# Autodesk Inventor assembly: TestAssem
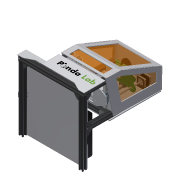
[picture p0: Inventor's stored thumbnail of the model, 180x180]
Saved by Autodesk Inventor 2014 (Build 180170000, 170)
## iProperties
Created: 2015-01-19
Part Number: TestAssem
Document SubType Name: Assembly
Designer: Peele
Author: Peele
## Documents named in this file (21)
- E:\Copy\DLP\PandaPrint\SubAssem\TestAssem.iam
- E:\Copy\DLP\PandaPrint\SubAssem\InnerTopAssem.iam
- E:\Copy\DLP\PandaPrint\SubAssem\NewVatAssem.iam
- E:\Copy\DLP\PandaPrint\CustomParts\InnerFront.ipt
- E:\Copy\DLP\PandaPrint\CustomParts\InnerSide.ipt
- E:\Copy\DLP\PandaPrint\SubAssem\NewFrame.iam
- E:\Copy\DLP\PandaPrint\CustomParts\ProjectorPlate.ipt
- E:\Copy\DLP\PandaPrint\StockParts\Projector-AcerP1500.ipt
- E:\Copy\DLP\PandaPrint\CustomParts\MirrorPlate.ipt
- E:\Copy\DLP\PandaPrint\SubAssem\StepperWithMount.iam
- E:\Copy\DLP\PandaPrint\CustomParts\BackPlate.ipt
- E:\Copy\DLP\PandaPrint\StockParts\Rail.ipt
- E:\Copy\DLP\PandaPrint\SubAssem\PlatformAssenm.iam
- E:\Copy\DLP\PandaPrint\StockParts\bLOCK.ipt
- E:\Copy\DLP\PandaPrint\CustomParts\BottomRightSide.ipt
- E:\Copy\DLP\PandaPrint\SubAssem\FrontCover.iam
- E:\Copy\DLP\PandaPrint\CustomParts\LeftSidePanel.ipt
- E:\Copy\DLP\PandaPrint\CustomParts\FrontPanel.ipt
- E:\Copy\DLP\PandaPrint\CustomParts\ControlRightPanel.ipt
- E:\Copy\DLP\PandaPrint\StockParts\Rail\Rail-02.ipt
- E:\Copy\DLP\PandaPrint\CustomParts\ControlPanel.ipt
## Components (21 placed, 19 different names)
1. InnerTopAssem:1 [sub-assembly] — Mate:1, Flush:1, Mate:2, Mate:3, Mate:4, Flush:2, Mate:5, Mate:10, Flush:7, Flush:13, Mate:27, Mate:31, Mate:44, Flush:28, Mate:49
2. NewVatAssem:1 [sub-assembly] — Mate:3, Mate:4, Mate:51
3. InnerFront:1 — Flush:2, Mate:5, Flush:12, Flush:7
4. NewFrame:1 [sub-assembly] — Mate:10, Flush:12, Mate:13, Flush:5, Flush:6, Flush:13, Mate:20, Flush:17, Flush:18, Mate:32, Flush:19, Flush:20, Mate:36, Flush:21, Flush:22, Flush:23, Mate:37, Mate:38, Flush:24, Mate:41, Flush:25, Flush:26, Mate:50
5. ProjectorPlate:1 — Mate:13, Flush:5, Flush:6, Mate:14, Mate:15
6. Projector-AcerP1500:1 — Mate:14
7. MirrorPlate:1 — Mate:15, Flush:17
8. StepperWithMount:1 [sub-assembly] — Mate:44, Mate:45
9. BackPlate:1 — Mate:20, Mate:21, Mate:40, Flush:25, Mate:45, Flush:26, Mate:46
10. Rail-02:1 — Mate:21, Mate:22, Mate:25, Mate:27
11. PlatformAssenm:1 [sub-assembly] — Mate:23, Mate:26, Mate:28, Mate:51
12. bLOCK:1 — Mate:22, Mate:23, Mate:25, Mate:26, Mate:28
13. StepperWithMount:2 [sub-assembly] — Mate:40
14. InnerSide:1 — Flush:18, Mate:31, Mate:32, Mate:33
15. BottomRightSide:1 — Mate:33, Flush:19, Flush:20
16. FrontCover:1 [sub-assembly] — Mate:41, Mate:46
17. LeftSidePanel:1 — Mate:36, Flush:21, Flush:22, Mate:47, Mate:48
18. FrontPanel:1 — Flush:23, Mate:37, Mate:43, Flush:27
19. ControlRightPanel:1 — Mate:38, Flush:24, Mate:43
20. ControlPanel:1 — Mate:47, Mate:48, Flush:27
21. InnerSide:2 — Flush:28, Mate:49, Mate:50
## Relationships (53: Mate 34, Flush 19)
- Mate:1: InnerTopAssem:1
- Flush:1: InnerTopAssem:1
- Mate:2: InnerTopAssem:1
- Mate:3: InnerTopAssem:1 ↔ NewVatAssem:1
- Mate:4: InnerTopAssem:1 ↔ NewVatAssem:1
- Flush:2: InnerTopAssem:1 ↔ InnerFront:1
- Mate:5: InnerTopAssem:1 ↔ InnerFront:1
- Mate:10: InnerTopAssem:1 ↔ NewFrame:1
- Flush:12: InnerFront:1 ↔ NewFrame:1
- Mate:13: NewFrame:1 ↔ ProjectorPlate:1
- Flush:5: NewFrame:1 ↔ ProjectorPlate:1
- Flush:6: NewFrame:1 ↔ ProjectorPlate:1
- Mate:14: ProjectorPlate:1 ↔ Projector-AcerP1500:1
- Mate:15: ProjectorPlate:1 ↔ MirrorPlate:1
- Flush:7: InnerTopAssem:1 ↔ InnerFront:1
- Flush:13: InnerTopAssem:1 ↔ NewFrame:1
- Mate:20: NewFrame:1 ↔ BackPlate:1
- Mate:21: BackPlate:1 ↔ Rail-02:1
- Mate:22: Rail-02:1 ↔ bLOCK:1
- Mate:23: PlatformAssenm:1 ↔ bLOCK:1
- Mate:25: Rail-02:1 ↔ bLOCK:1
- Mate:26: PlatformAssenm:1 ↔ bLOCK:1
- Mate:27: InnerTopAssem:1 ↔ Rail-02:1
- Mate:28: PlatformAssenm:1 ↔ bLOCK:1
- Flush:17 (85 mm): NewFrame:1 ↔ MirrorPlate:1
- Flush:18: NewFrame:1 ↔ InnerSide:1
- Mate:31: InnerTopAssem:1 ↔ InnerSide:1
- Mate:32: NewFrame:1 ↔ InnerSide:1
- Mate:33: InnerSide:1 ↔ BottomRightSide:1
- Flush:19: NewFrame:1 ↔ BottomRightSide:1
- Flush:20: NewFrame:1 ↔ BottomRightSide:1
- Mate:36: NewFrame:1 ↔ LeftSidePanel:1
- Flush:21: NewFrame:1 ↔ LeftSidePanel:1
- Flush:22: NewFrame:1 ↔ LeftSidePanel:1
- Flush:23: NewFrame:1 ↔ FrontPanel:1
- Mate:37: NewFrame:1 ↔ FrontPanel:1
- Mate:38: NewFrame:1 ↔ ControlRightPanel:1
- Flush:24: NewFrame:1 ↔ ControlRightPanel:1
- Mate:40: BackPlate:1 ↔ StepperWithMount:2
- Mate:41: NewFrame:1 ↔ FrontCover:1
- Flush:25: NewFrame:1 ↔ BackPlate:1
- Mate:43: FrontPanel:1 ↔ ControlRightPanel:1
- Mate:44: InnerTopAssem:1 ↔ StepperWithMount:1
- Mate:45: StepperWithMount:1 ↔ BackPlate:1
- Flush:26 (6 mm): NewFrame:1 ↔ BackPlate:1
- Mate:46: BackPlate:1 ↔ FrontCover:1
- Mate:47: LeftSidePanel:1 ↔ ControlPanel:1
- Mate:48: LeftSidePanel:1 ↔ ControlPanel:1
- Flush:27: FrontPanel:1 ↔ ControlPanel:1
- Flush:28: InnerTopAssem:1 ↔ InnerSide:2
- Mate:49: InnerTopAssem:1 ↔ InnerSide:2
- Mate:50: NewFrame:1 ↔ InnerSide:2
- Mate:51: NewVatAssem:1 ↔ PlatformAssenm:1
